# Autodesk Inventor assembly: additionalhand
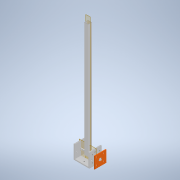
[picture p0: Inventor's stored thumbnail of the model, 180x180]
Saved by Autodesk Inventor 2022 (Build 260153000, 153)
## iProperties
Created: 2022-04-20
Part Number: additionalhand
Document SubType Name: Assembly
Designer: Yazawa
Author: Yazawa
## Documents named in this file (8)
- C:\Users\Yazawa\Documents\GitHub\University\minakatalab\shacho\additionalhand.iam
- C:\Users\Yazawa\Documents\GitHub\University\minakatalab\shacho\hand.ipt
- C:\Users\Yazawa\Documents\GitHub\University\minakatalab\shacho\Spacer10mm.ipt
- C:\Users\Yazawa\Documents\GitHub\University\minakatalab\shacho\pcb.ipt
- C:\Users\Yazawa\Documents\GitHub\University\minakatalab\shacho\FL674ZZ.ipt
- C:\Users\Yazawa\Documents\GitHub\University\minakatalab\shacho\shaft.ipt
- C:\Users\Yazawa\Documents\GitHub\University\minakatalab\shacho\stick.ipt
- C:\Users\Yazawa\Documents\GitHub\University\minakatalab\shacho\stopper.ipt
## Components (13 placed, 7 different names)
1. hand:1 — メイト:1, メイト:2, メイト:4, メイト:5, メイト:6, メイト:7, メイト:9, メイト:10, メイト:11, メイト:12, メイト:13, メイト:16, メイト:17, メイト:18, メイト:20, メイト:21, フラッシュ:1, メイト:25, メイト:26, フラッシュ:4, フラッシュ:5, フラッシュ:6, 角度:2
2. Spacer10mm:1 — メイト:6, メイト:7
3. Spacer10mm:2 — メイト:4, メイト:5
4. Spacer10mm:3 — メイト:9, メイト:10, メイト:14, メイト:15
5. Spacer10mm:4 — メイト:2, メイト:11
6. pcb:1 — メイト:12, メイト:14, メイト:15, メイト:19, メイト:22, フラッシュ:2
7. FL674ZZ:1 — メイト:19, メイト:22
8. FL674ZZ:2 — メイト:18, メイト:21
9. FL674ZZ:3 — メイト:17, メイト:20, メイト:23
10. shaft:1 — メイト:23, メイト:24, フラッシュ:3, フラッシュ:6, 角度:1
11. stick:1 — メイト:24, フラッシュ:5, 角度:1, 角度:2
12. stopper:1 — フラッシュ:1, メイト:25
13. stopper:2 — メイト:26, フラッシュ:4
## Relationships (32: Mate 24, Flush 6, Angle 2)
- メイト:1 [Mate]: hand:1
- メイト:2 [Mate]: hand:1 ↔ Spacer10mm:4
- メイト:4 [Mate]: hand:1 ↔ Spacer10mm:2
- メイト:5 [Mate]: hand:1 ↔ Spacer10mm:2
- メイト:6 [Mate]: hand:1 ↔ Spacer10mm:1
- メイト:7 [Mate]: hand:1 ↔ Spacer10mm:1
- メイト:9 [Mate]: hand:1 ↔ Spacer10mm:3
- メイト:10 [Mate]: hand:1 ↔ Spacer10mm:3
- メイト:11 [Mate]: hand:1 ↔ Spacer10mm:4
- メイト:12 [Mate]: hand:1 ↔ pcb:1
- メイト:13 [Mate]: hand:1
- メイト:14 [Mate]: Spacer10mm:3 ↔ pcb:1
- メイト:15 [Mate]: Spacer10mm:3 ↔ pcb:1
- メイト:16 [Mate]: hand:1
- メイト:17 [Mate]: hand:1 ↔ FL674ZZ:3
- メイト:18 [Mate]: hand:1 ↔ FL674ZZ:2
- メイト:19 [Mate]: pcb:1 ↔ FL674ZZ:1
- メイト:20 [Mate]: hand:1 ↔ FL674ZZ:3
- メイト:21 [Mate]: hand:1 ↔ FL674ZZ:2
- メイト:22 [Mate]: pcb:1 ↔ FL674ZZ:1
- メイト:23 [Mate]: FL674ZZ:3 ↔ shaft:1
- メイト:24 [Mate]: shaft:1 ↔ stick:1
- フラッシュ:1 [Flush]: hand:1 ↔ stopper:1
- フラッシュ:2 [Flush] (2 mm): pcb:1
- フラッシュ:3 [Flush]: shaft:1
- メイト:25 [Mate]: hand:1 ↔ stopper:1
- メイト:26 [Mate]: hand:1 ↔ stopper:2
- フラッシュ:4 [Flush]: hand:1 ↔ stopper:2
- フラッシュ:5 [Flush]: hand:1 ↔ stick:1
- フラッシュ:6 [Flush]: hand:1 ↔ shaft:1
- 角度:1 [Angle] (0 deg): shaft:1 ↔ stick:1
- 角度:2 [Angle] (0 deg): hand:1 ↔ stick:1
